# Autodesk Inventor assembly: Почти готово_CPY
(part 3 of 3)
- Жесткий:378 [WeldJoint]: Крышка фонаря 2_MIR_CPY:1 ↔ Болт ГОСТ Р 50274-92 M8-6g×16-F:193
- Жесткий:379 [WeldJoint]: Крышка фонаря 2_MIR_CPY:1 ↔ Болт ГОСТ Р 50274-92 M8-6g×16-F:194
- Жесткий:380 [WeldJoint]: Крышка фонаря 2_MIR_CPY:1 ↔ Болт ГОСТ Р 50274-92 M8-6g×16-F:195
- Жесткий:381 [WeldJoint]: Крышка фонаря 2_MIR_CPY:1 ↔ Болт ГОСТ Р 50274-92 M8-6g×16-F:196
- Жесткий:382 [WeldJoint]: Крышка фонаря 2_MIR_CPY:1 ↔ Болт ГОСТ Р 50274-92 M8-6g×16-F:197
- Жесткий:383 [WeldJoint]: Крышка фонаря 2_MIR_CPY:1 ↔ Болт ГОСТ Р 50274-92 M8-6g×16-F:198
- Жесткий:384 [WeldJoint]: Крышка фонаря 2_MIR_CPY:1 ↔ Болт ГОСТ Р 50274-92 M8-6g×16-F:199
- Жесткий:385 [WeldJoint]: Крышка фонаря 2_MIR_CPY:1 ↔ Болт ГОСТ Р 50274-92 M8-6g×16-F:200
- Жесткий:386 [WeldJoint]: Крышка фонаря 2_MIR_CPY:1 ↔ Болт ГОСТ Р 50274-92 M8-6g×16-F:201
- Жесткий:387 [WeldJoint]: Крышка фонаря 2_MIR_CPY:1 ↔ Болт ГОСТ Р 50274-92 M8-6g×16-F:202
- Жесткий:388 [WeldJoint]: Крышка фонаря 2_MIR_CPY:1 ↔ Болт ГОСТ Р 50274-92 M8-6g×16-F:203
- Жесткий:389 [WeldJoint]: Крышка фонаря 2_MIR_CPY:1 ↔ Болт ГОСТ Р 50274-92 M8-6g×16-F:204
- Жесткий:390 [WeldJoint]: Крышка фонаря 2_MIR_CPY:1 ↔ Болт ГОСТ Р 50274-92 M8-6g×16-F:205
- Жесткий:391 [WeldJoint]: Крышка фонаря 2_MIR_CPY:1 ↔ Болт ГОСТ Р 50274-92 M8-6g×16-F:206
- Жесткий:392 [WeldJoint]: Крышка фонаря 2_MIR_CPY:1 ↔ Болт ГОСТ Р 50274-92 M8-6g×16-F:207
- Жесткий:393 [WeldJoint]: Крышка фонаря 2_MIR_CPY:1 ↔ Болт ГОСТ Р 50274-92 M8-6g×16-F:208
- Жесткий:394 [WeldJoint]: Крышка фонаря 2_MIR_CPY:1 ↔ Болт ГОСТ Р 50274-92 M8-6g×16-F:209
- Жесткий:395 [WeldJoint]: Крышка фонаря 2_MIR_CPY:1 ↔ Болт ГОСТ Р 50274-92 M8-6g×16-F:210
- Жесткий:396 [WeldJoint]: Крышка фонаря 2_MIR_CPY:1 ↔ Болт ГОСТ Р 50274-92 M8-6g×16-F:211
- Жесткий:397 [WeldJoint]: Крышка фонаря 2_MIR_CPY:1 ↔ Болт ГОСТ Р 50274-92 M8-6g×16-F:212
- Жесткий:398 [WeldJoint]: Крышка фонаря 2_MIR_CPY:1 ↔ Болт ГОСТ Р 50274-92 M8-6g×16-F:213
- Жесткий:399 [WeldJoint]: Крышка фонаря 2_MIR_CPY:1 ↔ Болт ГОСТ Р 50274-92 M8-6g×16-F:214
- Жесткий:400 [WeldJoint]: Крышка фонаря 2_MIR_CPY:1 ↔ Болт ГОСТ Р 50274-92 M8-6g×16-F:215
- Жесткий:401 [WeldJoint]: Крышка фонаря 2_MIR_CPY:1 ↔ Болт ГОСТ Р 50274-92 M8-6g×16-F:216
- Жесткий:402 [WeldJoint]: Крышка фонаря 2_MIR_CPY:1 ↔ Болт ГОСТ Р 50274-92 M8-6g×16-F:217
- Жесткий:403 [WeldJoint]: Крышка фонаря 2_MIR_CPY:1 ↔ Болт ГОСТ Р 50274-92 M8-6g×16-F:218
- Жесткий:404 [WeldJoint] (298.75 mm): Шток_CPY:1 ↔ Маслоотражательное кольцо_CPY:1
